# Autodesk Inventor assembly: HexaDrone
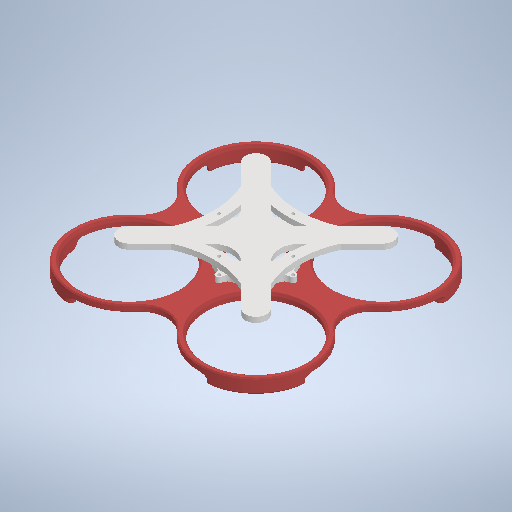
[picture p0: Inventor's stored thumbnail of the model, 512x512]
Saved by Autodesk Inventor 2025.1 (Build 291241020, 241B)
## iProperties
Created: 2024-09-22
Part Number: HexaDrone
Document SubType Name: Assembly
Designer: daare
Author: daare
## Documents named in this file (4)
- C:\Users\daare\Documents\Inventor\HexaDrone\HexaDrone.iam
- C:\Users\daare\Documents\Inventor\HexaDrone\Base.ipt
- C:\Users\daare\Documents\Inventor\HexaDrone\Frame.ipt
- C:\Users\daare\Documents\Inventor\HexaDrone\ModuleConnector.ipt
## Components (3 placed, 3 different names)
1. Base:1 — 메이트:1, 메이트:2, 각도:1, 메이트:3, 메이트:4, 메이트:17
2. Frame:1 — 메이트:3, 메이트:4, 메이트:14, 메이트:15, 메이트:16
3. ModuleConnector:1 — 메이트:14, 메이트:15, 메이트:16, 메이트:17
## Relationships (9: Mate 8, Angle 1)
- 메이트:1 [Mate]: Base:1
- 메이트:2 [Mate]: Base:1
- 각도:1 [Angle] (0 deg): Base:1
- 메이트:3 [Mate]: Base:1 ↔ Frame:1
- 메이트:4 [Mate]: Base:1 ↔ Frame:1
- 메이트:14 [Mate]: Frame:1 ↔ ModuleConnector:1
- 메이트:15 [Mate]: Frame:1 ↔ ModuleConnector:1
- 메이트:16 [Mate]: Frame:1 ↔ ModuleConnector:1
- 메이트:17 [Mate]: Base:1 ↔ ModuleConnector:1
